# Autodesk Inventor assembly: Portal-Column-v2
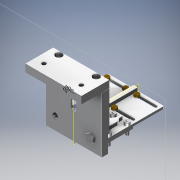
[picture p0: Inventor's stored thumbnail of the model, 180x180]
Saved by Autodesk Inventor 2016 (Build 200138000, 138)
## iProperties
Created: 2015-10-23
Part Number: Portal-Column-v2
Document SubType Name: Assembly
Designer: as
Author: as
## Documents named in this file (8)
- C:\Users\as\Documents\Inventor\mintplacer-export\export\Portal-Column-v2.iam
- C:\Users\as\Documents\Inventor\mintplacer-export\export\Portal-Column-v2-base.ipt
- C:\Users\as\Documents\Inventor\mintplacer-export\export\Portal-Column-v2-Column.ipt
- C:\Users\as\Documents\Inventor\mintplacer-export\export\Portal-Column-v2\Design Accelerator\Bolted Connection1.iam
- C:\Users\as\Documents\Inventor\Content Center Files\R2016\en-US\ISO 1207(1)\DIN EN ISO 1207 - M3 x 10.ipt
- C:\Users\as\Documents\Inventor\Content Center Files\R2016\en-US\ISO 4762(1)\DIN EN ISO 4762 - M3 x 10.ipt
- C:\Users\as\Documents\Inventor\mintplacer-export\export\Portal-Column-v2-Top.ipt
- C:\Users\as\Documents\Inventor\mintplacer-export\export\belt-clamp-15mm-htd.ipt
## Components (19 placed, 7 different names)
1. Portal-Column-v2-base:1 — Flush:1, Mate:2, Mate:3, Mate:4, Mate:5, Mate:6, Mate:7, Mate:8, Mate:9, Mate:10, Mate:11, Mate:12, Mate:15, Mate:16, Mate:19, Mate:20, Mate:21, Mate:22, Mate:23, Mate:24, Mate:25, Mate:26, Mate:27, Mate:28, Mate:29, Mate:30, Mate:31, Mate:32, Mate:33, Mate:34
2. Portal-Column-v2-Column:1 — Flush:1, Mate:1, Flush:2
3. M5 sides:1 [sub-assembly] — Mate:1, Mate:2
4. DIN EN ISO 1207 M3 x 10:1 — Mate:3, Mate:4
5. DIN EN ISO 1207 M3 x 10:2 — Mate:5, Mate:6
6. DIN EN ISO 1207 M3 x 10:3 — Mate:7, Mate:8
7. DIN EN ISO 1207 M3 x 10:4 — Mate:9, Mate:10
8. DIN EN ISO 1207 M3 x 10:5 — Mate:11, Mate:12
9. DIN EN ISO 1207 M3 x 10:7 — Mate:15, Mate:16
10. DIN EN ISO 4762 M3 x 10:1 — Mate:19, Mate:20
11. DIN EN ISO 4762 M3 x 10:2 — Mate:21, Mate:22
12. DIN EN ISO 4762 M3 x 10:3 — Mate:23, Mate:24
13. DIN EN ISO 4762 M3 x 10:4 — Mate:25, Mate:26
14. DIN EN ISO 4762 M3 x 10:5 — Mate:27, Mate:28
15. DIN EN ISO 4762 M3 x 10:6 — Mate:29, Mate:30
16. DIN EN ISO 4762 M3 x 10:7 — Mate:31, Mate:32
17. DIN EN ISO 4762 M3 x 10:8 — Mate:33, Mate:34
18. Portal-Column-v2-Top:1 — Flush:2
19. belt-clamp-15mm-htd:1
## Relationships (32: Mate 30, Flush 2)
- Flush:1 (-1.5 mm): Portal-Column-v2-base:1 ↔ Portal-Column-v2-Column:1
- Mate:1: Portal-Column-v2-Column:1 ↔ M5 sides:1
- Mate:2: Portal-Column-v2-base:1 ↔ M5 sides:1
- Mate:3: Portal-Column-v2-base:1 ↔ DIN EN ISO 1207 M3 x 10:1
- Mate:4: Portal-Column-v2-base:1 ↔ DIN EN ISO 1207 M3 x 10:1
- Mate:5: Portal-Column-v2-base:1 ↔ DIN EN ISO 1207 M3 x 10:2
- Mate:6: Portal-Column-v2-base:1 ↔ DIN EN ISO 1207 M3 x 10:2
- Mate:7: Portal-Column-v2-base:1 ↔ DIN EN ISO 1207 M3 x 10:3
- Mate:8: Portal-Column-v2-base:1 ↔ DIN EN ISO 1207 M3 x 10:3
- Mate:9: Portal-Column-v2-base:1 ↔ DIN EN ISO 1207 M3 x 10:4
- Mate:10: Portal-Column-v2-base:1 ↔ DIN EN ISO 1207 M3 x 10:4
- Mate:11: Portal-Column-v2-base:1 ↔ DIN EN ISO 1207 M3 x 10:5
- Mate:12: Portal-Column-v2-base:1 ↔ DIN EN ISO 1207 M3 x 10:5
- Mate:15: Portal-Column-v2-base:1 ↔ DIN EN ISO 1207 M3 x 10:7
- Mate:16: Portal-Column-v2-base:1 ↔ DIN EN ISO 1207 M3 x 10:7
- Mate:19: Portal-Column-v2-base:1 ↔ DIN EN ISO 4762 M3 x 10:1
- Mate:20: Portal-Column-v2-base:1 ↔ DIN EN ISO 4762 M3 x 10:1
- Mate:21: Portal-Column-v2-base:1 ↔ DIN EN ISO 4762 M3 x 10:2
- Mate:22: Portal-Column-v2-base:1 ↔ DIN EN ISO 4762 M3 x 10:2
- Mate:23: Portal-Column-v2-base:1 ↔ DIN EN ISO 4762 M3 x 10:3
- Mate:24: Portal-Column-v2-base:1 ↔ DIN EN ISO 4762 M3 x 10:3
- Mate:25: Portal-Column-v2-base:1 ↔ DIN EN ISO 4762 M3 x 10:4
- Mate:26: Portal-Column-v2-base:1 ↔ DIN EN ISO 4762 M3 x 10:4
- Mate:27: Portal-Column-v2-base:1 ↔ DIN EN ISO 4762 M3 x 10:5
- Mate:28: Portal-Column-v2-base:1 ↔ DIN EN ISO 4762 M3 x 10:5
- Mate:29: Portal-Column-v2-base:1 ↔ DIN EN ISO 4762 M3 x 10:6
- Mate:30: Portal-Column-v2-base:1 ↔ DIN EN ISO 4762 M3 x 10:6
- Mate:31: Portal-Column-v2-base:1 ↔ DIN EN ISO 4762 M3 x 10:7
- Mate:32: Portal-Column-v2-base:1 ↔ DIN EN ISO 4762 M3 x 10:7
- Mate:33: Portal-Column-v2-base:1 ↔ DIN EN ISO 4762 M3 x 10:8
- Mate:34: Portal-Column-v2-base:1 ↔ DIN EN ISO 4762 M3 x 10:8
- Flush:2: Portal-Column-v2-Column:1 ↔ Portal-Column-v2-Top:1
